# Autodesk Inventor assembly: crossAssembly
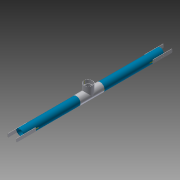
[picture p0: Inventor's stored thumbnail of the model, 180x180]
Saved by Autodesk Inventor 2014 (Build 180170000, 170)
## iProperties
Created: 2013-12-03
Part Number: crossAssembly
Document SubType Name: Assembly
Designer: Dave
Author: Dave
## Documents named in this file (4)
- C:\Users\ddeboer\Desktop\hera-cad\surface\crossAssembly.iam
- C:\Users\ddeboer\Desktop\hera-cad\smallParts\pvc_T_2in.ipt
- C:\Users\ddeboer\Desktop\hera-cad\surface\cross.ipt
- C:\Users\ddeboer\Desktop\hera-cad\smallParts\joinerBracket.ipt
## Components (7 placed, 3 different names)
1. pvc_T_2in:1 — Insert:2, Insert:3, Angle:2, Angle:3
2. cross:1 — Insert:2, Angle:3, Insert:5, Angle:4, Insert:7
3. cross:2 — Insert:3, Insert:4, Angle:1, Angle:2, Insert:6
4. joinerBracket:1 — Insert:4, Angle:1, Angle:5
5. joinerBracket:2 — Insert:6, Angle:5
6. joinerBracket:3 — Insert:7, Angle:6
7. joinerBracket:4 — Insert:5, Angle:4, Angle:6
## Relationships (12: Insert 6, Angle 6)
- Insert:2 (-25.4 mm): pvc_T_2in:1 ↔ cross:1
- Insert:3: pvc_T_2in:1 ↔ cross:2
- Insert:4: cross:2 ↔ joinerBracket:1
- Angle:1 (180 deg): cross:2 ↔ joinerBracket:1
- Angle:2 (0 deg): pvc_T_2in:1 ↔ cross:2
- Angle:3 (0 deg): pvc_T_2in:1 ↔ cross:1
- Insert:5: cross:1 ↔ joinerBracket:4
- Angle:4 (180 deg): cross:1 ↔ joinerBracket:4
- Insert:6: cross:2 ↔ joinerBracket:2
- Angle:5 (0 deg): joinerBracket:1 ↔ joinerBracket:2
- Insert:7: cross:1 ↔ joinerBracket:3
- Angle:6 (0 deg): joinerBracket:3 ↔ joinerBracket:4
